# Autodesk Inventor assembly: ArmWithBase
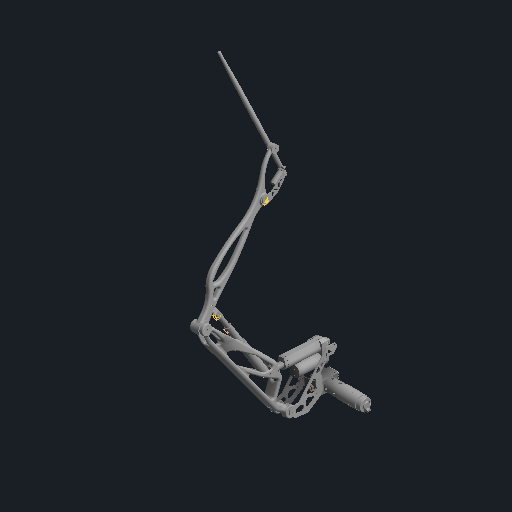
[picture p0: Inventor's stored thumbnail of the model, 512x512]
Saved by Autodesk Inventor 2025.2 (Build 292293000, 293)
## iProperties
Created: 2025-01-19
Part Number: ArmWithBase
Document SubType Name: Assembly
Designer: valer
Author: valer
## Documents named in this file (3)
- C:\Users\valer\Desktop\str1ker\cad\ArmWithBase.iam
- C:\Users\valer\Desktop\str1ker\cad\ArmBase.iam
- C:\Users\valer\Desktop\str1ker\cad\Arm.iam
## Components (2 placed, 2 different names)
1. Base:1 [sub-assembly] — Mate:4, Mate:5, Mate:6, Mate:7
2. Arm:1 [sub-assembly] — Mate:5, Mate:6, Mate:8
## Relationships (5: Mate 5)
- Mate:4: Base:1
- Mate:5: Base:1 ↔ Arm:1
- Mate:6: Base:1 ↔ Arm:1
- Mate:7: Base:1
- Mate:8: Arm:1
